# Autodesk Inventor assembly: Smart Orbiter Mockup - Right Angle Mount
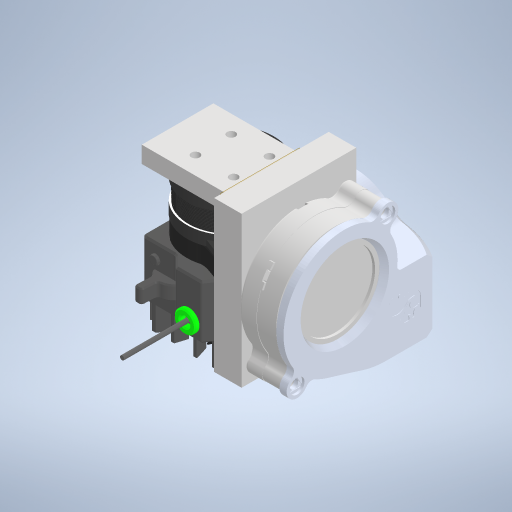
[picture p0: Inventor's stored thumbnail of the model, 512x512]
Saved by Autodesk Inventor 2023 (Build 270158000, 158)
## iProperties
Created: 2024-03-07
Part Number: Smart Orbiter Mockup - Right Angle Mount
Document SubType Name: Assembly
Designer: AdminForWorker
Title: Smart Orbiter Mockup v1
Author: AdminForWorker
## Documents named in this file (13)
- C:\Users\incep\OneDrive\Desktop\3D Printer Stuff\Smart Orbiter V3 Design for Sigmax\Smart Orbiter Mockup - Right Angle Mount.iam
- C:\Users\incep\OneDrive\Desktop\3D Printer Stuff\Smart Orbiter V3 Design for Sigmax\FilamentCoupler.iam
- C:\Users\incep\OneDrive\Desktop\3D Printer Stuff\Smart Orbiter V3 Design for Sigmax\FAN .iam
- C:\Users\incep\OneDrive\Desktop\3D Printer Stuff\Smart Orbiter V3 Design for Sigmax\HeatSink.ipt
- C:\Users\incep\OneDrive\Desktop\3D Printer Stuff\Smart Orbiter V3 Design for Sigmax\HuBHousing.ipt
- C:\Users\incep\OneDrive\Desktop\3D Printer Stuff\Smart Orbiter V3 Design for Sigmax\Electronics.iam
- C:\Users\incep\OneDrive\Desktop\3D Printer Stuff\Smart Orbiter V3 Design for Sigmax\LDO_36STH17-1004AHG v6 v1.iam
- C:\Users\incep\OneDrive\Desktop\3D Printer Stuff\Smart Orbiter V3 Design for Sigmax\Orbiter Gearset.iam
- C:\Users\incep\OneDrive\Desktop\3D Printer Stuff\Smart Orbiter V3 Design for Sigmax\Nuts&Bolts.iam
- C:\Users\incep\OneDrive\Desktop\3D Printer Stuff\Smart Orbiter V3 Design for Sigmax\Heatblock.iam
- C:\Users\incep\OneDrive\Desktop\3D Printer Stuff\Sigmax-Orbiter-Adapter-Plate-Right Angle.ipt
- C:\Users\incep\OneDrive\Desktop\3D Printer Stuff\Smart Orbiter V3 Design for Sigmax\Smart Orbiter v3 - duct.ipt
- C:\Users\incep\OneDrive\Desktop\3D Printer Stuff\Smart Orbiter V3 Design for Sigmax\BFB0512HH-F00.ipt
## Components (12 placed, 12 different names)
1. FilamentCoupler:1 [sub-assembly]
2. FAN :1 [sub-assembly]
3. HeatSink:1 — Mate:1, Mate:2, Angle:1
4. HuBHousing:1
5. Electronics:1 [sub-assembly]
6. LDO_36STH17-1004AHG v6 v1:1 [sub-assembly]
7. Orbiter Gearset:1 [sub-assembly]
8. Nuts&Bolts:1 [sub-assembly]
9. Heatblock:1 [sub-assembly]
10. Sigmax-Orbiter-Adapter-Plate-Right Angle:1 — Mate:1, Mate:2, Angle:1, Mate:3, Mate:4, Mate:5
11. Smart Orbiter v3 - duct:1 — Mate:6, Mate:7, Mate:8
12. BFB0512HH-F00:1 — Mate:3, Mate:4, Mate:5, Mate:6, Mate:7, Mate:8
## Relationships (9: Mate 8, Angle 1)
- Mate:1: HeatSink:1 ↔ Sigmax-Orbiter-Adapter-Plate-Right Angle:1
- Mate:2: HeatSink:1 ↔ Sigmax-Orbiter-Adapter-Plate-Right Angle:1
- Angle:1 (0 deg): HeatSink:1 ↔ Sigmax-Orbiter-Adapter-Plate-Right Angle:1
- Mate:3: Sigmax-Orbiter-Adapter-Plate-Right Angle:1 ↔ BFB0512HH-F00:1
- Mate:4: Sigmax-Orbiter-Adapter-Plate-Right Angle:1 ↔ BFB0512HH-F00:1
- Mate:5: Sigmax-Orbiter-Adapter-Plate-Right Angle:1 ↔ BFB0512HH-F00:1
- Mate:6: Smart Orbiter v3 - duct:1 ↔ BFB0512HH-F00:1
- Mate:7: Smart Orbiter v3 - duct:1 ↔ BFB0512HH-F00:1
- Mate:8: Smart Orbiter v3 - duct:1 ↔ BFB0512HH-F00:1
